# Autodesk Inventor assembly: Assembly1
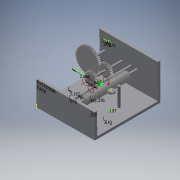
[picture p0: Inventor's stored thumbnail of the model, 180x180]
Saved by Autodesk Inventor 2017 (Build 210142000, 142)
## iProperties
Created: 2019-10-30
Part Number: Assembly1
Document SubType Name: Assembly
Designer: Manan
Author: Manan
## Documents named in this file (10)
- C:\Users\Manan\OneDrive\Desktop\EXAM\Assembly1.iam
- C:\Users\Manan\OneDrive\Desktop\ENG 1C03\Submission\GIVEN - SpurGearMount (2).ipt
- C:\Users\Manan\OneDrive\Desktop\ENG 1C03\Submission\GIVEN - ShortRod (2).ipt
- C:\Users\Manan\OneDrive\Desktop\EXAM\Assembly1\Design Accelerator\Spur Gears2.iam
- C:\Users\Manan\OneDrive\Desktop\EXAM\Medium rod.ipt
- C:\Users\Manan\OneDrive\Desktop\EXAM\Assembly1\Design Accelerator\Spur Gears3.iam
- C:\Users\Manan\OneDrive\Desktop\EXAM\GIVEN - LongRod (2).ipt
- C:\Users\Manan\OneDrive\Desktop\EXAM\Assembly1\Design Accelerator\Spur Gears4.iam
- C:\Users\Manan\OneDrive\Desktop\EXAM\GIVEN - WormDriveMount (2).ipt
- C:\Users\Manan\OneDrive\Desktop\EXAM\Assembly1\Design Accelerator\Worm Gears15.iam
## Components (10 placed, 7 different names)
1. GIVEN - SpurGearMount (2):1 — Flush:1, Mate:1, Mate:3, Flush:3, Mate:6, Flush:5, Flush:6, Mate:9, Flush:9
2. GIVEN - ShortRod (2):1 — Flush:1, Mate:1, Mate:2, Flush:2
3. Spur Gears:2 [sub-assembly] — Mate:2, Flush:2, Mate:4
4. Medium rod:1 — Mate:3, Flush:3, Mate:4, Mate:5, Flush:4
5. Spur Gears:3 [sub-assembly] — Mate:5, Flush:4
6. GIVEN - LongRod (2):1 — Mate:6, Flush:5, Mate:7, Flush:7, Mate:8, Flush:8
7. Spur Gears:4 [sub-assembly] — Mate:7, Flush:6, Flush:7
8. GIVEN - WormDriveMount (2):1 — Mate:8, Flush:8, Flush:10, Angle:1
9. Worm Gears:2 [sub-assembly] — Mate:10, Flush:10, Angle:1
10. GIVEN - LongRod (2):2 — Mate:9, Flush:9, Mate:10
## Relationships (21: Flush 10, Mate 10, Angle 1)
- Flush:1: GIVEN - SpurGearMount (2):1 ↔ GIVEN - ShortRod (2):1
- Mate:1: GIVEN - SpurGearMount (2):1 ↔ GIVEN - ShortRod (2):1
- Mate:2: GIVEN - ShortRod (2):1 ↔ Spur Gears:2
- Flush:2: GIVEN - ShortRod (2):1 ↔ Spur Gears:2
- Mate:3: GIVEN - SpurGearMount (2):1 ↔ Medium rod:1
- Flush:3: GIVEN - SpurGearMount (2):1 ↔ Medium rod:1
- Mate:4: Spur Gears:2 ↔ Medium rod:1
- Mate:5: Medium rod:1 ↔ Spur Gears:3
- Flush:4: Medium rod:1 ↔ Spur Gears:3
- Mate:6: GIVEN - SpurGearMount (2):1 ↔ GIVEN - LongRod (2):1
- Flush:5: GIVEN - SpurGearMount (2):1 ↔ GIVEN - LongRod (2):1
- Mate:7: GIVEN - LongRod (2):1 ↔ Spur Gears:4
- Flush:6 (70 mm): GIVEN - SpurGearMount (2):1 ↔ Spur Gears:4
- Flush:7: GIVEN - LongRod (2):1 ↔ Spur Gears:4
- Mate:8: GIVEN - LongRod (2):1 ↔ GIVEN - WormDriveMount (2):1
- Flush:8: GIVEN - LongRod (2):1 ↔ GIVEN - WormDriveMount (2):1
- Mate:9: GIVEN - SpurGearMount (2):1 ↔ GIVEN - LongRod (2):2
- Flush:9: GIVEN - SpurGearMount (2):1 ↔ GIVEN - LongRod (2):2
- Mate:10: Worm Gears:2 ↔ GIVEN - LongRod (2):2
- Flush:10 (20 mm): GIVEN - WormDriveMount (2):1 ↔ Worm Gears:2
- Angle:1 (0 deg): GIVEN - WormDriveMount (2):1 ↔ Worm Gears:2
